# Autodesk Inventor assembly: SHOT_1_002_ShooterAssembly
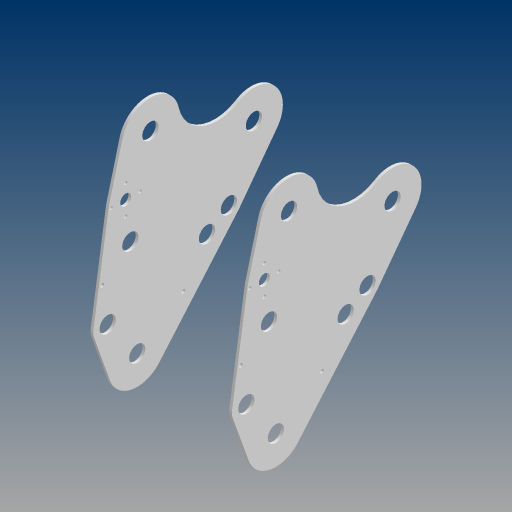
[picture p0: Inventor's stored thumbnail of the model, 512x512]
Saved by Autodesk Inventor 2024.3 (Build 283343000, 343)
## iProperties
Created: 2024-08-07
Part Number: SHOT_1_002_ShooterAssembly
Document SubType Name: Assembly
Designer: Kenji
Author: Kenji
## Documents named in this file (2)
- C:\Users\Kenji\Documents\GitHub\1622-2024-Summer-CAD-A-Thon\Shooter\SHOT_1_002_ShooterAssembly.iam
- C:\Users\Kenji\Documents\GitHub\1622-2024-Summer-CAD-A-Thon\Shooter\SHOT_1_001_ShooterPlate.ipt
## Components (2 placed, 1 different names)
1. SHOT_1_001_ShooterPlate:1 — Mate:1, Mate:2
2. SHOT_1_001_ShooterPlate:2 — Mate:1, Mate:2
## Relationships (2: Mate 2)
- Mate:1: SHOT_1_001_ShooterPlate:1 ↔ SHOT_1_001_ShooterPlate:2
- Mate:2: SHOT_1_001_ShooterPlate:1 ↔ SHOT_1_001_ShooterPlate:2
